# Autodesk Inventor assembly: ARM
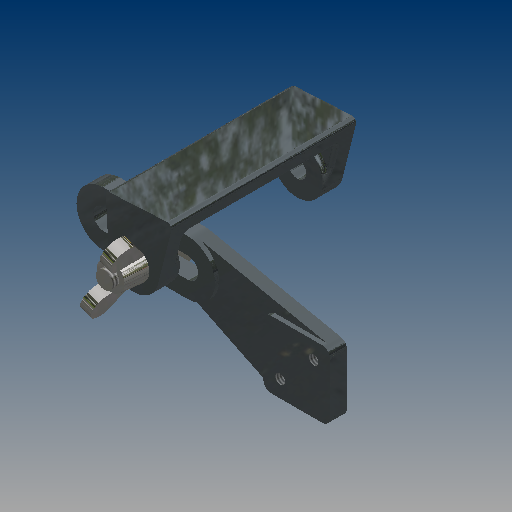
[picture p0: Inventor's stored thumbnail of the model, 512x512]
Saved by Autodesk Inventor 2020 (Build 240168000, 168)
## iProperties
Created: 2019-11-15
Part Number: ARM
Document SubType Name: Assembly
Designer: Jorge
Author: Jorge
## Documents named in this file (5)
- C:\Users\gerar\OneDrive - Instituto Tecnologico y de Estudios Superiores de Monterrey\TEC\Semestre XI\Dibujo Computarizado\Archivos de Inventor\Esmeril\ARM\ARM.iam
- C:\Users\gerar\OneDrive - Instituto Tecnologico y de Estudios Superiores de Monterrey\TEC\Semestre XI\Dibujo Computarizado\Archivos de Inventor\Esmeril\ARM\ToolRestarm.ipt
- C:\Users\gerar\OneDrive - Instituto Tecnologico y de Estudios Superiores de Monterrey\TEC\Semestre XI\Dibujo Computarizado\Archivos de Inventor\Esmeril\ARM\ANSI B18.17 - 1_4 - 20B (1).ipt
- C:\Users\gerar\OneDrive - Instituto Tecnologico y de Estudios Superiores de Monterrey\TEC\Semestre XI\Dibujo Computarizado\Archivos de Inventor\Esmeril\ARM\ANSI B18.5 - 1_4-20 UNC - 1(6).ipt
- C:\Users\gerar\OneDrive - Instituto Tecnologico y de Estudios Superiores de Monterrey\TEC\Semestre XI\Dibujo Computarizado\Archivos de Inventor\Esmeril\ARM\ToolRest.ipt
## Components (4 placed, 4 different names)
1. ToolRestarm:1 — Mate:5, Tangent:1, Mate:7, Transitional:1
2. ToolRest:1 — Mate:5, Mate:6, Mate:9
3. Round Head Bolt - Inch 1/4-20 UNC - 1:1 — Tangent:1, Mate:6, Mate:7, Mate:8, Transitional:1
4. Type B - Style 1 - Wing Nut - Inch 1/4 - 20:1 — Mate:8, Mate:9
## Relationships (7: Mate 5, Tangent 1, Transitional 1)
- Mate:5: ToolRestarm:1 ↔ ToolRest:1
- Tangent:1: ToolRestarm:1 ↔ Round Head Bolt - Inch 1/4-20 UNC - 1:1
- Mate:6: ToolRest:1 ↔ Round Head Bolt - Inch 1/4-20 UNC - 1:1
- Mate:7: ToolRestarm:1 ↔ Round Head Bolt - Inch 1/4-20 UNC - 1:1
- Mate:8: Round Head Bolt - Inch 1/4-20 UNC - 1:1 ↔ Type B - Style 1 - Wing Nut - Inch 1/4 - 20:1
- Mate:9: ToolRest:1 ↔ Type B - Style 1 - Wing Nut - Inch 1/4 - 20:1
- Transitional:1: ToolRestarm:1 ↔ Round Head Bolt - Inch 1/4-20 UNC - 1:1
